# Autodesk Inventor assembly: 13042026
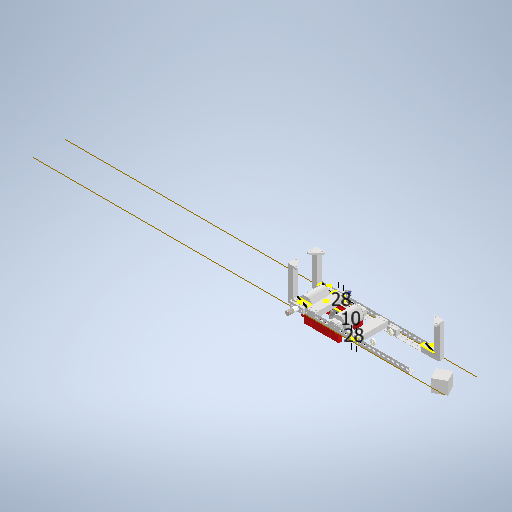
[picture p0: Inventor's stored thumbnail of the model, 512x512]
Saved by Autodesk Inventor 2025.2 (Build 292293000, 293)
## iProperties
Created: 2026-04-13
Part Number: 13042026
Document SubType Name: Assembly
Designer: Oski
Author: Oski
## Documents named in this file (21)
- C:\Users\Oski\Desktop\ProjektPrzejsciowy\Inventor\13042026\13042026.iam
- C:\Users\Oski\Desktop\ProjektPrzejsciowy\Inventor\13042026\Parts\28BYJ48 — kopia\28BYJ48 — kopia\28BYJ48 — kopia.ipt
- C:\Users\Oski\Desktop\ProjektPrzejsciowy\Inventor\13042026\Parts\13042025-02.ipt
- C:\Users\Oski\Desktop\ProjektPrzejsciowy\Inventor\13042026\Parts\706-2_6200ZZ_10x30x9mm_Groove_Ball_Bearing_STEP242\706-2_6200ZZ_10x30x9mm_Groove_Ball_Bearing_STEP242\706-2_6200ZZ_10x30x9mm_Groove_Ball_Bearing_.iam
- C:\Users\Oski\Desktop\ProjektPrzejsciowy\Inventor\13042026\Parts\706-2_6200ZZ_10x30x9mm_Groove_Ball_Bearing_STEP242\25d-metal-gearmotor-172-227\25d-metal-gearmotor-172-227\25d-metal-gearmotor-172-227.ipt
- C:\Users\Oski\Desktop\ProjektPrzejsciowy\Inventor\13042026\Parts\13042026-01.ipt
- C:\Users\Oski\Desktop\ProjektPrzejsciowy\Inventor\13042026\Parts\13042026-04.ipt
- C:\Users\Oski\Desktop\ProjektPrzejsciowy\Inventor\13042026\Parts\13042026-03.ipt
- C:\Users\Oski\Desktop\ProjektPrzejsciowy\Inventor\13042026\Parts\13042026-05.ipt
- C:\Users\Oski\Desktop\ProjektPrzejsciowy\Inventor\13042026\Parts\13042026-06.ipt
- C:\Users\Oski\Desktop\ProjektPrzejsciowy\Inventor\13042026\Parts\m8x40_din933.ipt
- C:\Users\Oski\Desktop\ProjektPrzejsciowy\Inventor\13042026\Parts\1883316.iam
- C:\Users\Oski\Desktop\ProjektPrzejsciowy\Inventor\13042026\Parts\13042026-07.ipt
- C:\Users\Oski\Desktop\ProjektPrzejsciowy\Inventor\13042026\Parts\13042026-09.ipt
- C:\Users\Oski\Desktop\ProjektPrzejsciowy\Inventor\13042026\Parts\13042026-08.ipt
- C:\Users\Oski\Desktop\ProjektPrzejsciowy\Inventor\13042026\Parts\13042026-14.ipt
- C:\Users\Oski\Desktop\ProjektPrzejsciowy\Inventor\13042026\Parts\13042026-12.ipt
- C:\Users\Oski\Desktop\ProjektPrzejsciowy\Inventor\13042026\Parts\13042026-13.ipt
- C:\Users\Oski\Desktop\ProjektPrzejsciowy\Inventor\13042026\Parts\13042026-15.ipt
- C:\Users\Oski\Desktop\ProjektPrzejsciowy\Inventor\13042026\Parts\BOX.ipt
- C:\Users\Oski\Desktop\ProjektPrzejsciowy\Inventor\13042026\Parts\13042026-16.ipt
## Components (40 placed, 20 different names)
1. 28BYJ48 — kopia:1 — Mate:107, Mate:108, Mate:109
2. 13042025-02:1 — Mate:103, Mate:104, Mate:107, Mate:109
3. 706-2_6200ZZ_10x30x9mm_Groove_Ball_Bearing_:1 [sub-assembly] — Insert:1, Rotational:2
4. 25d-metal-gearmotor-172-227:1 — Mate:19, Mate:20, Mate:21, Mate:22, Mate:23
5. 13042026-01:1 — Insert:1, Insert:3
6. 13042026-04:1 — Mate:24, Mate:28, Mate:29, Mate:30, Mate:31, Mate:32, Mate:45, Mate:60, Mate:61, Mate:62, Mate:66, Mate:67, Mate:68, Mate:73, Flush:1, Mate:82, Mate:85, Mate:86, Mate:87, Flush:2, Flush:3, Mate:94, Mate:95, Mate:96, Mate:97, Mate:98, Mate:99
7. 13042026-04:2 — Mate:6, Mate:7, Mate:8, Mate:9, Mate:10, Mate:11, Mate:13, Mate:48, Angle:1, Mate:59, Mate:63, Mate:64, Mate:65, Mate:71, Mate:79, Mate:80, Mate:83, Mate:84, Mate:88, Mate:89, Mate:100, Flush:4
8. 13042026-03:1 — Rotational:1, Mate:6, Mate:9, Mate:10, Mate:12, Mate:14
9. 706-2_6200ZZ_10x30x9mm_Groove_Ball_Bearing_:2 [sub-assembly] — Insert:3, Rotational:1
10. 13042026-03:2 — Rotational:2, Mate:73, Mate:92, Mate:93
11. 13042026-06:1 — Mate:7, Mate:8, Mate:110
12. m8x40_din933:1 — Mate:11, Mate:12
13. m8x40_din933:2 — Mate:13, Mate:14
14. 1883316:1 [sub-assembly] — Mate:17, Mate:18
15. 1883316:2 [sub-assembly] — Mate:15, Mate:16
16. 13042026-07:1 — Mate:15, Mate:16, Mate:17, Mate:18, Mate:24, Mate:28, Mate:29
17. 13042026-09:1 — Mate:19, Mate:20, Mate:21, Mate:30, Mate:31, Mate:32
18. 13042026-08:1 — Mate:22, Mate:23, Mate:77, Mate:78
19. 706-2_6200ZZ_10x30x9mm_Groove_Ball_Bearing_:3 [sub-assembly] — Mate:76
20. 13042026-01:2 — Mate:74, Mate:76
21. 13042026-03:3 — Mate:45, Mate:66, Mate:67
22. 706-2_6200ZZ_10x30x9mm_Groove_Ball_Bearing_:4 [sub-assembly] — Mate:74
23. 13042026-03:4 — Mate:48, Mate:65
24. 706-2_6200ZZ_10x30x9mm_Groove_Ball_Bearing_:5 [sub-assembly]
25. 13042026-03:5
26. 13042026-05:1 — Mate:68, Mate:71, Mate:87, Mate:88, Mate:89
27. 13042026-14:1 — Mate:77, Mate:78
28. 13042026-12:1 — Mate:59, Mate:63, Mate:64
29. 13042026-13:1 — Mate:60, Mate:61, Mate:62
30. 13042026-15:1 — Mate:79, Flush:3, Mate:99
31. 13042026-15:2 — Mate:80, Flush:2, Mate:98
32. BOX:1 — Mate:81
33. 13042026-05:2 — Mate:82, Mate:83, Mate:84, Mate:85, Mate:86, Mate:90, Mate:91
34. m8x40_din933:3 — Mate:90, Mate:97
35. m8x40_din933:4 — Mate:91, Mate:94
36. m8x40_din933:5 — Mate:92, Mate:95
37. m8x40_din933:6 — Mate:93, Mate:96
38. 13042026-16:1 — Mate:100, Flush:4, Mate:105, Mate:106, Mate:108, Mate:110
39. 1883316:3 [sub-assembly] — Mate:103, Mate:104, Mate:105, Mate:106
40. 28BYJ48 — kopia:2
## Relationships (84: Mate 72, RevoluteJoint 5, Flush 4, Insert 2, Angle 1)
- Insert:1: 706-2_6200ZZ_10x30x9mm_Groove_Ball_Bearing_:1 ↔ 13042026-01:1
- Insert:3: 13042026-01:1 ↔ 706-2_6200ZZ_10x30x9mm_Groove_Ball_Bearing_:2
- Rotational:1 [RevoluteJoint]: 13042026-03:1 ↔ 706-2_6200ZZ_10x30x9mm_Groove_Ball_Bearing_:2
- Rotational:2 [RevoluteJoint]: 706-2_6200ZZ_10x30x9mm_Groove_Ball_Bearing_:1 ↔ 13042026-03:2
- Mate:6: 13042026-04:2 ↔ 13042026-03:1
- Mate:7: 13042026-04:2 ↔ 13042026-06:1
- Mate:8: 13042026-04:2 ↔ 13042026-06:1
- Mate:9: 13042026-04:2 ↔ 13042026-03:1
- Mate:10: 13042026-04:2 ↔ 13042026-03:1
- Mate:11: 13042026-04:2 ↔ m8x40_din933:1
- Mate:12: 13042026-03:1 ↔ m8x40_din933:1
- Mate:13: 13042026-04:2 ↔ m8x40_din933:2
- Mate:14: 13042026-03:1 ↔ m8x40_din933:2
- Mate:15: 1883316:2 ↔ 13042026-07:1
- Mate:16: 1883316:2 ↔ 13042026-07:1
- Mate:17: 1883316:1 ↔ 13042026-07:1
- Mate:18: 1883316:1 ↔ 13042026-07:1
- Mate:19: 25d-metal-gearmotor-172-227:1 ↔ 13042026-09:1
- Mate:20: 25d-metal-gearmotor-172-227:1 ↔ 13042026-09:1
- Mate:21: 25d-metal-gearmotor-172-227:1 ↔ 13042026-09:1
- Mate:22: 25d-metal-gearmotor-172-227:1 ↔ 13042026-08:1
- Mate:23: 25d-metal-gearmotor-172-227:1 ↔ 13042026-08:1
- Mate:24: 13042026-04:1 ↔ 13042026-07:1
- Mate:28: 13042026-04:1 ↔ 13042026-07:1
- Mate:29: 13042026-04:1 ↔ 13042026-07:1
- Mate:30: 13042026-04:1 ↔ 13042026-09:1
- Mate:31: 13042026-04:1 ↔ 13042026-09:1
- Mate:32: 13042026-04:1 ↔ 13042026-09:1
- [RevoluteJoint]: 13042026-03:3 ↔ 706-2_6200ZZ_10x30x9mm_Groove_Ball_Bearing_:4
- [RevoluteJoint]: 706-2_6200ZZ_10x30x9mm_Groove_Ball_Bearing_:3 ↔ 13042026-03:4
- Mate:45: 13042026-04:1 ↔ 13042026-03:3
- Mate:48: 13042026-04:2 ↔ 13042026-03:4
- [RevoluteJoint]: 706-2_6200ZZ_10x30x9mm_Groove_Ball_Bearing_:5 ↔ 13042026-03:5
- Angle:1 (0 deg): 13042026-04:2
- Mate:59: 13042026-04:2 ↔ 13042026-12:1
- Mate:60: 13042026-04:1 ↔ 13042026-13:1
- Mate:61: 13042026-04:1 ↔ 13042026-13:1
- Mate:62: 13042026-04:1 ↔ 13042026-13:1
- Mate:63: 13042026-04:2 ↔ 13042026-12:1
- Mate:64: 13042026-04:2 ↔ 13042026-12:1
- Mate:65: 13042026-04:2 ↔ 13042026-03:4
- Mate:66: 13042026-04:1 ↔ 13042026-03:3
- Mate:67: 13042026-04:1 ↔ 13042026-03:3
- Mate:68: 13042026-04:1 ↔ 13042026-05:1
- Mate:71: 13042026-04:2 ↔ 13042026-05:1
- Mate:73: 13042026-04:1 ↔ 13042026-03:2
- Mate:74: 13042026-01:2 ↔ 706-2_6200ZZ_10x30x9mm_Groove_Ball_Bearing_:4
- Mate:76: 706-2_6200ZZ_10x30x9mm_Groove_Ball_Bearing_:3 ↔ 13042026-01:2
- Mate:77: 13042026-08:1 ↔ 13042026-14:1
- Mate:78: 13042026-08:1 ↔ 13042026-14:1
- Mate:79: 13042026-04:2 ↔ 13042026-15:1
- Mate:80: 13042026-04:2 ↔ 13042026-15:2
- Mate:81: BOX:1
- Flush:1 (-20.5 mm): 13042026-04:1
- Mate:82: 13042026-04:1 ↔ 13042026-05:2
- Mate:83: 13042026-04:2 ↔ 13042026-05:2
- Mate:84: 13042026-04:2 ↔ 13042026-05:2
- Mate:85: 13042026-04:1 ↔ 13042026-05:2
- Mate:86: 13042026-04:1 ↔ 13042026-05:2
- Mate:87: 13042026-04:1 ↔ 13042026-05:1
- Mate:88: 13042026-04:2 ↔ 13042026-05:1
- Mate:89: 13042026-04:2 ↔ 13042026-05:1
- Mate:90: 13042026-05:2 ↔ m8x40_din933:3
- Mate:91: 13042026-05:2 ↔ m8x40_din933:4
- Mate:92: 13042026-03:2 ↔ m8x40_din933:5
- Mate:93: 13042026-03:2 ↔ m8x40_din933:6
- Flush:2: 13042026-04:1 ↔ 13042026-15:2
- Flush:3: 13042026-04:1 ↔ 13042026-15:1
- Mate:94: 13042026-04:1 ↔ m8x40_din933:4
- Mate:95: 13042026-04:1 ↔ m8x40_din933:5
- Mate:96: 13042026-04:1 ↔ m8x40_din933:6
- Mate:97: 13042026-04:1 ↔ m8x40_din933:3
- Mate:98: 13042026-04:1 ↔ 13042026-15:2
- Mate:99: 13042026-04:1 ↔ 13042026-15:1
- Mate:100: 13042026-04:2 ↔ 13042026-16:1
- Mate:103: 13042025-02:1 ↔ 1883316:3
- Mate:104: 13042025-02:1 ↔ 1883316:3
- Flush:4: 13042026-04:2 ↔ 13042026-16:1
- Mate:105: 13042026-16:1 ↔ 1883316:3
- Mate:106: 13042026-16:1 ↔ 1883316:3
- Mate:107: 28BYJ48 — kopia:1 ↔ 13042025-02:1
- Mate:108: 28BYJ48 — kopia:1 ↔ 13042026-16:1
- Mate:109: 28BYJ48 — kopia:1 ↔ 13042025-02:1
- Mate:110: 13042026-06:1 ↔ 13042026-16:1
## Named parameters: d77_d6 = 0 mm, d78_d7 = -154.125091 deg, d79_d8 = 0 mm, d80_d9 = 73.789448 deg, d85_d8 = 0 mm, d86_d9 = -101.748209 deg, Finish1_Area = 1019.55, Finish1_Thickness = 0.05 mm, Finish2_Area = 185.373, Finish2_Thickness = 0.05 mm
note: some values were not read from the file. Shown as the stored number, unit unknown: "Finish1_Area", "Finish2_Area".
